# Autodesk Inventor assembly: Telescope
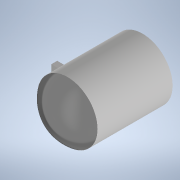
[picture p0: Inventor's stored thumbnail of the model, 180x180]
Saved by Autodesk Inventor 2022 (Build 260153000, 153)
## iProperties
Created: 2023-08-20
Part Number: Telescope
Document SubType Name: Assembly
Designer: fouad
Author: fouad
## Documents named in this file (4)
- C:\Users\fouad\Documents\Telescope\Telescope.iam
- C:\Users\fouad\Documents\Telescope\Aperture.ipt
- C:\Users\fouad\Documents\Telescope\Main Mirror, f=24mm.ipt
- C:\Users\fouad\Documents\Telescope\Viewing Mirror.ipt
## Components (3 placed, 3 different names)
1. Aperture:1 — Mate:1, Mate:2, Rigid:1, Mate:3, Angle:1
2. Main Mirror, f=24mm:1 — Mate:1, Mate:2
3. Viewing Mirror:1 — Rigid:1
## Relationships (5: Mate 3, WeldJoint 1, Angle 1)
- Mate:1: Aperture:1 ↔ Main Mirror, f=24mm:1
- Mate:2: Aperture:1 ↔ Main Mirror, f=24mm:1
- Rigid:1 [WeldJoint]: Aperture:1 ↔ Viewing Mirror:1
- Mate:3: Aperture:1
- Angle:1 (90 deg): Aperture:1
